# Autodesk Inventor assembly: Version1Model
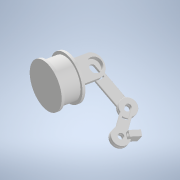
[picture p0: Inventor's stored thumbnail of the model, 180x180]
Saved by Autodesk Inventor 2022 (Build 260153000, 153)
## iProperties
Created: 2022-01-28
Part Number: Version1Model
Document SubType Name: Assembly
Designer: Alexa
Author: Alexa
## Documents named in this file (6)
- C:\Users\Alexa\Documents\4TH YEAR\Version1Model.iam
- C:\Users\Alexa\Documents\4TH YEAR\Other\new base.ipt
- C:\Users\Alexa\Documents\4TH YEAR\Other\Base Top.ipt
- C:\Users\Alexa\Documents\4TH YEAR\Other\First arm.ipt
- C:\Users\Alexa\Documents\4TH YEAR\Other\2nd arm.ipt
- C:\Users\Alexa\Documents\4TH YEAR\Other\End motor link.ipt
## Components (5 placed, 5 different names)
1. new base:1 — Rotational:1
2. Base Top:1 — Rotational:1, Rotational:4
3. First arm:1 — Rotational:4, Rotational:5
4. 2nd arm:1 — Rotational:5, Rotational:6
5. End motor link:1 — Rotational:6
## Relationships (4: RevoluteJoint 4)
- Rotational:1 [RevoluteJoint]: new base:1 ↔ Base Top:1
- Rotational:4 [RevoluteJoint]: Base Top:1 ↔ First arm:1
- Rotational:5 [RevoluteJoint]: First arm:1 ↔ 2nd arm:1
- Rotational:6 [RevoluteJoint]: 2nd arm:1 ↔ End motor link:1
